# Autodesk Inventor assembly: 組合1
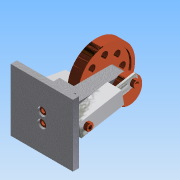
[picture p0: Inventor's stored thumbnail of the model, 180x180]
Saved by Autodesk Inventor 2015 (Build 190159000, 159)
## iProperties
Created: 2019-09-24
Part Number: 組合1
Document SubType Name: Assembly
Designer: d8910
Author: d8910
## Documents named in this file (11)
- C:\Users\d8910\Desktop\組合1.iam
- C:\Users\d8910\Desktop\零件3.ipt
- C:\Users\d8910\Desktop\零件1.ipt
- C:\Users\d8910\Desktop\零件5.ipt
- C:\Users\d8910\Desktop\零件2.ipt
- C:\Users\d8910\Desktop\零件4.ipt
- C:\Users\d8910\Desktop\零件6.ipt
- C:\Users\d8910\Desktop\零件7.ipt
- C:\Users\d8910\Desktop\DIN 6912 - M5 x 30.ipt
- C:\Users\d8910\Desktop\DIN 6912 - M5 x 12.ipt
- C:\Users\d8910\Desktop\DIN 6912 - M5 x 10.ipt
## Components (16 placed, 10 different names)
1. 零件3:1 — 貼合:1, 貼合:2, 貼合:3, 貼合:7, 插入:10, 插入:11, 角度:1
2. 零件1:1 — 貼合:4, 貼合:5, 貼合:7, 插入:1, 貼合:19, 貼合:24, 貼合:29
3. 零件5:1 — 貼合:10, 插入:2, 插入:3, 貼合:14, 角度:1
4. 零件2:1 — 貼合:17, 貼合:18, 插入:6
5. 零件2:2 — 貼合:25, 貼合:26, 插入:7
6. 零件4:1 — 貼合:22, 插入:5, 貼合:27, 插入:9
7. 零件4:2 — 插入:4, 貼合:16, 插入:12
8. 零件6:1 — 插入:1, 貼合:9, 插入:2, 貼合:15, 插入:4
9. 零件7:1 — 貼合:12, 插入:3, 貼合:14, 貼合:15, 貼合:23, 插入:5, 插入:8
10. DIN 6912 - M5 x 30:1 — 插入:6
11. DIN 6912 - M5 x 30:2 — 插入:7
12. DIN 6912 - M5 x 12:1 — 插入:10
13. DIN 6912 - M5 x 12:2 — 插入:11
14. DIN 6912 - M5 x 12:4 — 插入:8
15. DIN 6912 - M5 x 12:5 — 插入:9
16. DIN 6912 - M5 x 10:1 — 插入:12
## Relationships (42: Mate 29, Insert 12, Angle 1)
- 貼合:1 [Mate]: 零件3:1
- 貼合:2 [Mate]: 零件3:1
- 貼合:3 [Mate]: 零件3:1
- 貼合:4 [Mate]: 零件1:1
- 貼合:5 [Mate]: 零件1:1
- 貼合:6 [Mate]
- 貼合:7 [Mate]: 零件3:1 ↔ 零件1:1
- 貼合:8 [Mate]
- 插入:1 [Insert]: 零件1:1 ↔ 零件6:1
- 貼合:9 [Mate]: 零件6:1
- 貼合:10 [Mate]: 零件5:1
- 貼合:11 [Mate]
- 插入:2 [Insert]: 零件5:1 ↔ 零件6:1
- 貼合:12 [Mate]: 零件7:1
- 貼合:13 [Mate]
- 插入:3 [Insert]: 零件5:1 ↔ 零件7:1
- 貼合:14 [Mate]: 零件5:1 ↔ 零件7:1
- 貼合:15 [Mate]: 零件6:1 ↔ 零件7:1
- 插入:4 [Insert]: 零件4:2 ↔ 零件6:1
- 貼合:16 [Mate]: 零件4:2
- 貼合:17 [Mate]: 零件2:1
- 貼合:18 [Mate]: 零件2:1
- 貼合:19 [Mate]: 零件1:1
- 貼合:20 [Mate]
- 貼合:21 [Mate]
- 貼合:22 [Mate]: 零件4:1
- 貼合:23 [Mate]: 零件7:1
- 貼合:24 [Mate]: 零件1:1
- 貼合:25 [Mate]: 零件2:2
- 貼合:26 [Mate]: 零件2:2
- 插入:5 [Insert]: 零件4:1 ↔ 零件7:1
- 貼合:27 [Mate]: 零件4:1
- 貼合:28 [Mate]
- 貼合:29 [Mate]: 零件1:1
- 插入:6 [Insert]: 零件2:1 ↔ DIN 6912 - M5 x 30:1
- 插入:7 [Insert]: 零件2:2 ↔ DIN 6912 - M5 x 30:2
- 插入:8 [Insert]: 零件7:1 ↔ DIN 6912 - M5 x 12:4
- 插入:9 [Insert]: 零件4:1 ↔ DIN 6912 - M5 x 12:5
- 插入:10 [Insert]: 零件3:1 ↔ DIN 6912 - M5 x 12:1
- 插入:11 [Insert]: 零件3:1 ↔ DIN 6912 - M5 x 12:2
- 插入:12 [Insert]: 零件4:2 ↔ DIN 6912 - M5 x 10:1
- 角度:1 [Angle] (1080 deg): 零件3:1 ↔ 零件5:1
